# Autodesk Inventor assembly: complete
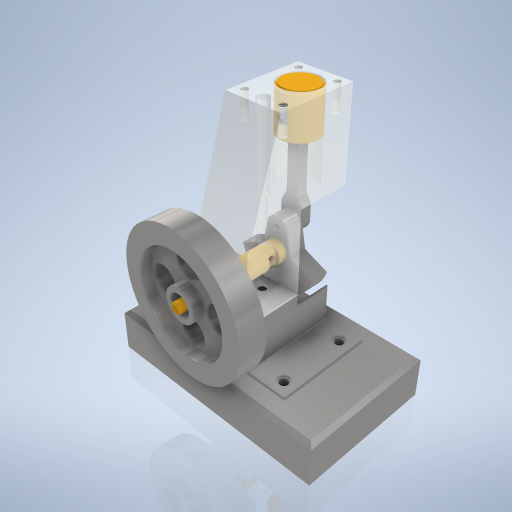
[picture p0: Inventor's stored thumbnail of the model, 512x512]
Saved by Autodesk Inventor 2024.2 (Build 282272000, 272)
## iProperties
Created: 2024-04-07
Part Number: complete
Document SubType Name: Assembly
Designer: Fabri
Author: Fabri
## Documents named in this file (8)
- C:\Users\Fabri\Documents\Inventor\Durckluft\complete.iam
- C:\Users\Fabri\Documents\Inventor\Durckluft\Grundplatte.ipt
- C:\Users\Fabri\Documents\Inventor\Durckluft\Bügelbefestigung.ipt
- C:\Users\Fabri\Documents\Inventor\Durckluft\MotorBlock.ipt
- C:\Users\Fabri\Documents\Inventor\Durckluft\inner_body.iam
- C:\Users\Fabri\Documents\Inventor\Durckluft\Kurbel.ipt
- C:\Users\Fabri\Documents\Inventor\Durckluft\Kurbelwelle.ipt
- C:\Users\Fabri\Documents\Inventor\Durckluft\Schwungscheibe.ipt
## Components (7 placed, 7 different names)
1. Grundplatte:1 — Passend:1
2. Bügelbefestigung:1 — Passend:1, Einfügen:1
3. MotorBlock:1 — Einfügen:1, Einfügen:2
4. inner_body:1 [sub-assembly] — Einfügen:2, Einfügen:3
5. Kurbel:1 — Einfügen:3, Einfügen:4
6. Kurbelwelle:1 — Einfügen:4, Passend:2
7. Schwungscheibe:1 — Passend:2
## Relationships (6: Insert 4, Mate 2)
- Passend:1 [Mate]: Grundplatte:1 ↔ Bügelbefestigung:1
- Einfügen:1 [Insert]: Bügelbefestigung:1 ↔ MotorBlock:1
- Einfügen:2 [Insert] (-32 mm): MotorBlock:1 ↔ inner_body:1
- Einfügen:3 [Insert]: inner_body:1 ↔ Kurbel:1
- Einfügen:4 [Insert] (-34 mm): Kurbel:1 ↔ Kurbelwelle:1
- Passend:2 [Mate]: Kurbelwelle:1 ↔ Schwungscheibe:1
